# Autodesk Inventor assembly: byk
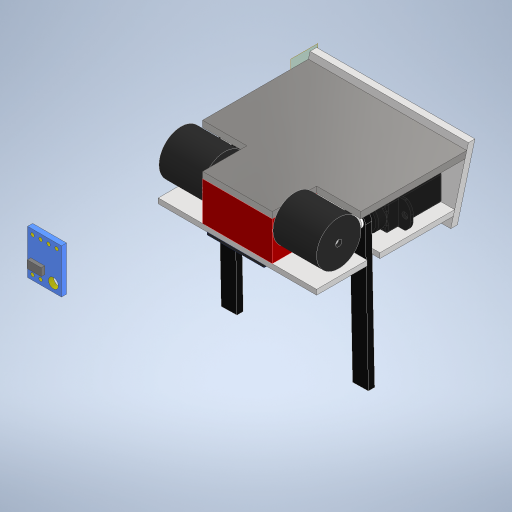
[picture p0: Inventor's stored thumbnail of the model, 512x512]
Saved by Autodesk Inventor 2023 (Build 270158000, 158)
## iProperties
Created: 2023-07-30
Part Number: byk
Document SubType Name: Assembly
Designer: Kamil
Author: Kamil
## Documents named in this file (13)
- C:\Users\Kamil\Documents\Inventor\MikroNalesnik\byk.iam
- C:\Users\Kamil\Documents\Inventor\MikroNalesnik\silnik_2.ipt
- C:\Users\Kamil\Documents\Inventor\MikroNalesnik\spod.ipt
- C:\Users\Kamil\Documents\Inventor\MikroNalesnik\TOF_VL53L0X (1).ipt
- C:\Users\Kamil\Documents\Inventor\MikroNalesnik\servo_mini_1370hd_cos.ipt
- C:\Users\Kamil\Documents\Inventor\MikroNalesnik\kolko.ipt
- C:\Users\Kamil\Documents\Inventor\MikroNalesnik\wach.ipt
- C:\Users\Kamil\Documents\Inventor\MikroNalesnik\uchwyt silnikow.ipt
- C:\Users\Kamil\Documents\Inventor\MikroNalesnik\PCB_BYK.ipt
- C:\Users\Kamil\Documents\Inventor\MikroNalesnik\ESP32-C3-WROOM-02.ipt
- C:\Users\Kamil\Documents\Inventor\MikroNalesnik\li-pol 35x30x4.ipt
- C:\Users\Kamil\Documents\Inventor\MikroNalesnik\pcb.ipt
- C:\Users\Kamil\Documents\Inventor\MikroNalesnik\noz.ipt
## Components (17 placed, 12 different names)
1. silnik_2:2 — Zestawiające:21, Zestawiające:23, Zestawiające:25, Zestawiające:26, Zestawiające:27
2. spod:1 — Zestawiające:10, Zestawiające:11, Równoległe:7, Równoległe:8, Zestawiające:22, Zestawiające:24, Równoległe:9, Równoległe:23, Kątowe:1, Równoległe:27, Zestawiające:33, Równoległe:28
3. servo_mini_1370hd_cos:1 — Zestawiające:10, Równoległe:5, Równoległe:8, Zestawiające:18, Zestawiające:19
4. servo_mini_1370hd_cos:2 — Zestawiające:11, Równoległe:5, Zestawiające:16, Zestawiające:17, Równoległe:7, Zestawiające:30
5. kolko:1
6. wach:1 — Zestawiające:16, Zestawiające:17
7. wach:2 — Zestawiające:18, Zestawiające:19
8. silnik_2:3 — Zestawiające:21, Zestawiające:22, Zestawiające:23
9. kolko:2 — Zestawiające:26, Zestawiające:27
10. uchwyt silnikow:1 — Zestawiające:24, Zestawiające:25, Równoległe:9, Równoległe:19, Zestawiające:31, Równoległe:24
11. PCB_BYK:1 — Równoległe:19
12. ESP32-C3-WROOM-02:1 — Zestawiające:32, Równoległe:26
13. li-pol 35x30x4:2 — Zestawiające:30, Równoległe:23, Zestawiające:31
14. pcb:1 — Równoległe:24, Zestawiające:32, Równoległe:26
15. TOF_VL53L0X (1):1 — Kątowe:1, Równoległe:27, Zestawiające:33
16. noz:1 — Równoległe:28
17. TOF_VL53L0X (1):2
## Relationships (28: Mate 17, Flush 10, Angle 1)
- Zestawiające:10 [Mate]: spod:1 ↔ servo_mini_1370hd_cos:1
- Zestawiające:11 [Mate]: spod:1 ↔ servo_mini_1370hd_cos:2
- Równoległe:5 [Flush]: servo_mini_1370hd_cos:1 ↔ servo_mini_1370hd_cos:2
- Zestawiające:16 [Mate]: servo_mini_1370hd_cos:2 ↔ wach:1
- Zestawiające:17 [Mate]: servo_mini_1370hd_cos:2 ↔ wach:1
- Równoległe:7 [Flush]: spod:1 ↔ servo_mini_1370hd_cos:2
- Równoległe:8 [Flush]: spod:1 ↔ servo_mini_1370hd_cos:1
- Zestawiające:18 [Mate]: servo_mini_1370hd_cos:1 ↔ wach:2
- Zestawiające:19 [Mate]: servo_mini_1370hd_cos:1 ↔ wach:2
- Zestawiające:21 [Mate] (2 mm): silnik_2:2 ↔ silnik_2:3
- Zestawiające:22 [Mate]: spod:1 ↔ silnik_2:3
- Zestawiające:23 [Mate]: silnik_2:2 ↔ silnik_2:3
- Zestawiające:24 [Mate]: spod:1 ↔ uchwyt silnikow:1
- Zestawiające:25 [Mate]: silnik_2:2 ↔ uchwyt silnikow:1
- Równoległe:9 [Flush]: spod:1 ↔ uchwyt silnikow:1
- Zestawiające:26 [Mate]: silnik_2:2 ↔ kolko:2
- Zestawiające:27 [Mate]: silnik_2:2 ↔ kolko:2
- Równoległe:19 [Flush]: uchwyt silnikow:1 ↔ PCB_BYK:1
- Zestawiające:30 [Mate]: servo_mini_1370hd_cos:2 ↔ li-pol 35x30x4:2
- Równoległe:23 [Flush] (10 mm): spod:1 ↔ li-pol 35x30x4:2
- Zestawiające:31 [Mate]: uchwyt silnikow:1 ↔ li-pol 35x30x4:2
- Równoległe:24 [Flush]: uchwyt silnikow:1 ↔ pcb:1
- Zestawiające:32 [Mate]: ESP32-C3-WROOM-02:1 ↔ pcb:1
- Równoległe:26 [Flush]: ESP32-C3-WROOM-02:1 ↔ pcb:1
- Kątowe:1 [Angle] (190 deg): spod:1 ↔ TOF_VL53L0X (1):1
- Równoległe:27 [Flush]: spod:1 ↔ TOF_VL53L0X (1):1
- Zestawiające:33 [Mate]: spod:1 ↔ TOF_VL53L0X (1):1
- Równoległe:28 [Flush]: spod:1 ↔ noz:1
